# Autodesk Inventor assembly: ForkMountWithBevelGear
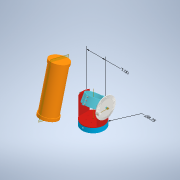
[picture p0: Inventor's stored thumbnail of the model, 180x180]
Saved by Autodesk Inventor 2021 (Build 250183000, 183)
## iProperties
Created: 2020-06-16
Part Number: ForkMountWithBevelGear
Document SubType Name: Assembly
Designer: robst
Author: robst
## Documents named in this file (13)
- C:\git\CAD-Development\robSteele\ShapeWays\TelescopeProjects\TelescopeMount\ForkMountWithBevelGear.iam
- C:\git\CAD-Development\robSteele\ShapeWays\TelescopeProjects\TelescopeMount\ForkMountWithBevelGear\Design Accelerator\Bevel Gears4.iam
- C:\git\CAD-Development\robSteele\ShapeWays\TelescopeProjects\TelescopeMount\topOfRaBase.ipt
- C:\git\CAD-Development\robSteele\ShapeWays\TelescopeProjects\TelescopeMount\baseForBevelGearMount.ipt
- C:\git\CAD-Development\robSteele\ShapeWays\TelescopeProjects\TelescopeMount\10x3_8-keyedDriveShaft.ipt
- C:\git\CAD-Development\robSteele\ShapeWays\TelescopeProjects\TelescopeMount\raHandController.ipt
- C:\git\CAD-Development\robSteele\ShapeWays\TelescopeProjects\TelescopeMount\telescopeTube.ipt
- C:\git\CAD-Development\robSteele\ShapeWays\TelescopeProjects\TelescopeMount\tubeBracket.ipt
- C:\Users\robst\Documents\Inventor\Content Center Files\R2021\en-US\ANSI B18.21.1\ANSI B18.21.1 - 0.25.ipt
- C:\Users\robst\Documents\Inventor\Content Center Files\R2021\en-US\ANSI B18.22.1\ANSI B18.22.1 - 1_4 - narrow - Type A.ipt
- C:\Users\robst\Documents\Inventor\Content Center Files\R2021\en-US\ANSI B18.3(03)\ANSI B18.3 - 1_4-20 UNC - UNC - 1.25(1).ipt
- C:\Users\robst\Documents\Inventor\Content Center Files\R2021\en-US\IFI 100 107(2)\IFI 100_107 - 1_4 - 20 Metal Type.ipt
- C:\git\CAD-Development\robSteele\ShapeWays\TelescopeProjects\TelescopeMount\ForkMountWithBevelGear\Design Accelerator\Bevel Gears1.iam
## Components (39 placed, 11 different names)
1. topOfRaBase:1 — Insert:1, Insert:2, Insert:3, Insert:26
2. Bevel Gears:1 [sub-assembly] — Insert:1, Insert:2, Insert:4
3. baseForBevelGearMount:1 — Insert:3
4. 10x3_8-keyedDriveShaft:1 — Insert:4, Insert:5
5. raHandController:1 — Insert:5
6. telescopeTube:1
7. tubeBracket:1 — Flush:1, Mate:1, Mate:2, Mate:3, Mate:4, Mate:5, Mate:6, Mate:7, Mate:8, Mate:9, Mate:10, Mate:11, Mate:12, Mate:13, Mate:15, Mate:17, Mate:19, Mate:21, Mate:23
8. tubeBracket:2 — Flush:1, Mate:14, Mate:16, Mate:18, Mate:20, Mate:22, Mate:24, Insert:26, Insert:27, Mate:25
9. Helical Spring Lock Washers 0.25:1 — Mate:1, Mate:2, Insert:8
10. Plain Washer (Inch) 1/4 - narrow - Type A:1 — Insert:8, Insert:14
11. Plain Washer (Inch) 1/4 - narrow - Type A:2 — Insert:14, Insert:20
12. Hexagon Socket Button Head Cap Screw - Inch 1/4 - 20 x 1 1/4:1 — Insert:20
13. Prevailing Torque Type Hex Nut - Inch (IFI) 1/4 - 20 Metal Type:1 — Mate:13, Mate:14
14. Helical Spring Lock Washers 0.25:2 — Mate:3, Mate:4, Insert:9
15. Helical Spring Lock Washers 0.25:3 — Mate:5, Mate:6, Insert:10
16. Helical Spring Lock Washers 0.25:4 — Mate:7, Mate:8, Insert:11
17. Helical Spring Lock Washers 0.25:5 — Mate:9, Mate:10, Insert:12
18. Helical Spring Lock Washers 0.25:6 — Mate:11, Mate:12, Insert:13
19. Plain Washer (Inch) 1/4 - narrow - Type A:3 — Insert:9, Insert:15
20. Plain Washer (Inch) 1/4 - narrow - Type A:4 — Insert:10, Insert:16
21. Plain Washer (Inch) 1/4 - narrow - Type A:5 — Insert:11, Insert:17
22. Plain Washer (Inch) 1/4 - narrow - Type A:6 — Insert:12, Insert:18
23. Plain Washer (Inch) 1/4 - narrow - Type A:7 — Insert:13, Insert:19
24. Plain Washer (Inch) 1/4 - narrow - Type A:8 — Insert:15, Insert:21
25. Plain Washer (Inch) 1/4 - narrow - Type A:9 — Insert:16, Insert:22
26. Plain Washer (Inch) 1/4 - narrow - Type A:10 — Insert:17, Insert:23
27. Plain Washer (Inch) 1/4 - narrow - Type A:11 — Insert:18, Insert:24
28. Plain Washer (Inch) 1/4 - narrow - Type A:12 — Insert:19, Insert:25
29. Hexagon Socket Button Head Cap Screw - Inch 1/4 - 20 x 1 1/4:2 — Insert:21
30. Hexagon Socket Button Head Cap Screw - Inch 1/4 - 20 x 1 1/4:3 — Insert:22
31. Hexagon Socket Button Head Cap Screw - Inch 1/4 - 20 x 1 1/4:4 — Insert:23
32. Hexagon Socket Button Head Cap Screw - Inch 1/4 - 20 x 1 1/4:5 — Insert:24
33. Hexagon Socket Button Head Cap Screw - Inch 1/4 - 20 x 1 1/4:6 — Insert:25
34. Prevailing Torque Type Hex Nut - Inch (IFI) 1/4 - 20 Metal Type:2 — Mate:15, Mate:16
35. Prevailing Torque Type Hex Nut - Inch (IFI) 1/4 - 20 Metal Type:3 — Mate:17, Mate:18
36. Prevailing Torque Type Hex Nut - Inch (IFI) 1/4 - 20 Metal Type:4 — Mate:19, Mate:20
37. Prevailing Torque Type Hex Nut - Inch (IFI) 1/4 - 20 Metal Type:5 — Mate:21, Mate:22
38. Prevailing Torque Type Hex Nut - Inch (IFI) 1/4 - 20 Metal Type:6 — Mate:23, Mate:24
39. Bevel Gears:2 [sub-assembly] — Insert:27, Mate:25
## Relationships (51: Insert 25, Mate 25, Flush 1)
- Insert:1: topOfRaBase:1 ↔ Bevel Gears:1
- Insert:2: topOfRaBase:1 ↔ Bevel Gears:1
- Insert:3: topOfRaBase:1 ↔ baseForBevelGearMount:1
- Insert:4 (50.8 mm): Bevel Gears:1 ↔ 10x3_8-keyedDriveShaft:1
- Insert:5: 10x3_8-keyedDriveShaft:1 ↔ raHandController:1
- Flush:1: tubeBracket:1 ↔ tubeBracket:2
- Mate:1: tubeBracket:1 ↔ Helical Spring Lock Washers 0.25:1
- Mate:2: tubeBracket:1 ↔ Helical Spring Lock Washers 0.25:1
- Mate:3: tubeBracket:1 ↔ Helical Spring Lock Washers 0.25:2
- Mate:4: tubeBracket:1 ↔ Helical Spring Lock Washers 0.25:2
- Mate:5: tubeBracket:1 ↔ Helical Spring Lock Washers 0.25:3
- Mate:6: tubeBracket:1 ↔ Helical Spring Lock Washers 0.25:3
- Mate:7: tubeBracket:1 ↔ Helical Spring Lock Washers 0.25:4
- Mate:8: tubeBracket:1 ↔ Helical Spring Lock Washers 0.25:4
- Mate:9: tubeBracket:1 ↔ Helical Spring Lock Washers 0.25:5
- Mate:10: tubeBracket:1 ↔ Helical Spring Lock Washers 0.25:5
- Mate:11: tubeBracket:1 ↔ Helical Spring Lock Washers 0.25:6
- Mate:12: tubeBracket:1 ↔ Helical Spring Lock Washers 0.25:6
- Insert:8: Helical Spring Lock Washers 0.25:1 ↔ Plain Washer (Inch) 1/4 - narrow - Type A:1
- Insert:9: Helical Spring Lock Washers 0.25:2 ↔ Plain Washer (Inch) 1/4 - narrow - Type A:3
- Insert:10: Helical Spring Lock Washers 0.25:3 ↔ Plain Washer (Inch) 1/4 - narrow - Type A:4
- Insert:11: Helical Spring Lock Washers 0.25:4 ↔ Plain Washer (Inch) 1/4 - narrow - Type A:5
- Insert:12: Helical Spring Lock Washers 0.25:5 ↔ Plain Washer (Inch) 1/4 - narrow - Type A:6
- Insert:13: Helical Spring Lock Washers 0.25:6 ↔ Plain Washer (Inch) 1/4 - narrow - Type A:7
- Insert:14: Plain Washer (Inch) 1/4 - narrow - Type A:1 ↔ Plain Washer (Inch) 1/4 - narrow - Type A:2
- Insert:15: Plain Washer (Inch) 1/4 - narrow - Type A:3 ↔ Plain Washer (Inch) 1/4 - narrow - Type A:8
- Insert:16: Plain Washer (Inch) 1/4 - narrow - Type A:4 ↔ Plain Washer (Inch) 1/4 - narrow - Type A:9
- Insert:17: Plain Washer (Inch) 1/4 - narrow - Type A:5 ↔ Plain Washer (Inch) 1/4 - narrow - Type A:10
- Insert:18: Plain Washer (Inch) 1/4 - narrow - Type A:6 ↔ Plain Washer (Inch) 1/4 - narrow - Type A:11
- Insert:19: Plain Washer (Inch) 1/4 - narrow - Type A:7 ↔ Plain Washer (Inch) 1/4 - narrow - Type A:12
- Insert:20: Plain Washer (Inch) 1/4 - narrow - Type A:2 ↔ Hexagon Socket Button Head Cap Screw - Inch 1/4 - 20 x 1 1/4:1
- Insert:21: Plain Washer (Inch) 1/4 - narrow - Type A:8 ↔ Hexagon Socket Button Head Cap Screw - Inch 1/4 - 20 x 1 1/4:2
- Insert:22: Plain Washer (Inch) 1/4 - narrow - Type A:9 ↔ Hexagon Socket Button Head Cap Screw - Inch 1/4 - 20 x 1 1/4:3
- Insert:23: Plain Washer (Inch) 1/4 - narrow - Type A:10 ↔ Hexagon Socket Button Head Cap Screw - Inch 1/4 - 20 x 1 1/4:4
- Insert:24: Plain Washer (Inch) 1/4 - narrow - Type A:11 ↔ Hexagon Socket Button Head Cap Screw - Inch 1/4 - 20 x 1 1/4:5
- Insert:25: Plain Washer (Inch) 1/4 - narrow - Type A:12 ↔ Hexagon Socket Button Head Cap Screw - Inch 1/4 - 20 x 1 1/4:6
- Mate:13: tubeBracket:1 ↔ Prevailing Torque Type Hex Nut - Inch (IFI) 1/4 - 20 Metal Type:1
- Mate:14: tubeBracket:2 ↔ Prevailing Torque Type Hex Nut - Inch (IFI) 1/4 - 20 Metal Type:1
- Mate:15: tubeBracket:1 ↔ Prevailing Torque Type Hex Nut - Inch (IFI) 1/4 - 20 Metal Type:2
- Mate:16: tubeBracket:2 ↔ Prevailing Torque Type Hex Nut - Inch (IFI) 1/4 - 20 Metal Type:2
- Mate:17: tubeBracket:1 ↔ Prevailing Torque Type Hex Nut - Inch (IFI) 1/4 - 20 Metal Type:3
- Mate:18: tubeBracket:2 ↔ Prevailing Torque Type Hex Nut - Inch (IFI) 1/4 - 20 Metal Type:3
- Mate:19: tubeBracket:1 ↔ Prevailing Torque Type Hex Nut - Inch (IFI) 1/4 - 20 Metal Type:4
- Mate:20: tubeBracket:2 ↔ Prevailing Torque Type Hex Nut - Inch (IFI) 1/4 - 20 Metal Type:4
- Mate:21: tubeBracket:1 ↔ Prevailing Torque Type Hex Nut - Inch (IFI) 1/4 - 20 Metal Type:5
- Mate:22: tubeBracket:2 ↔ Prevailing Torque Type Hex Nut - Inch (IFI) 1/4 - 20 Metal Type:5
- Mate:23: tubeBracket:1 ↔ Prevailing Torque Type Hex Nut - Inch (IFI) 1/4 - 20 Metal Type:6
- Mate:24: tubeBracket:2 ↔ Prevailing Torque Type Hex Nut - Inch (IFI) 1/4 - 20 Metal Type:6
- Insert:26 (-38.1 mm): topOfRaBase:1 ↔ tubeBracket:2
- Insert:27: tubeBracket:2 ↔ Bevel Gears:2
- Mate:25: tubeBracket:2 ↔ Bevel Gears:2
